# Autodesk Inventor assembly: Vacubot v1
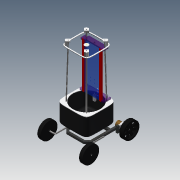
[picture p0: Inventor's stored thumbnail of the model, 180x180]
Saved by Autodesk Inventor 2014 SP1 (Build 180222100, 222)
## iProperties
Created: 2013-12-26
Part Number: Vacubot v1
Document SubType Name: Assembly
Designer: tom
Author: tom
## Documents named in this file (15)
- C:\Users\tom\Documents\GitHub\Vacubot\Inventor\Vacubot v1.iam
- C:\Users\tom\Documents\GitHub\Vacubot\Inventor\Base.ipt
- C:\Users\tom\Documents\GitHub\Vacubot\Inventor\Base Plate.ipt
- C:\Users\tom\Documents\GitHub\Vacubot\Inventor\Wheel Original.iam
- C:\Users\tom\Documents\GitHub\Vacubot\Inventor\Wheel Original_MIR.iam
- C:\Users\tom\Documents\GitHub\Vacubot\Inventor\GearMotor_Wheel.iam
- C:\Users\tom\Documents\GitHub\Vacubot\Inventor\GearMotor_Wheel_MIR.iam
- C:\Users\tom\Documents\GitHub\Vacubot\Inventor\Frame Lower.ipt
- C:\Users\tom\Documents\GitHub\Vacubot\Inventor\Part1.ipt
- C:\Users\tom\Documents\GitHub\Vacubot\Inventor\Center Rod.ipt
- C:\Users\tom\Documents\GitHub\Vacubot\Inventor\Upper Support.ipt
- C:\Users\tom\Documents\GitHub\Vacubot\Inventor\Lower Bracket.ipt
- C:\Users\tom\Documents\GitHub\Vacubot\Inventor\Gantry Motor.ipt
- C:\Users\tom\Documents\GitHub\Vacubot\Inventor\Z-table Rail.ipt
- C:\Users\tom\Documents\GitHub\Vacubot\Inventor\Z-table.ipt
## Components (18 placed, 14 different names)
1. Chassis — Mate:4, Mate:5, Mate:6
2. Base Plate:1 — Flush:1
3. Wheel Original:1 [sub-assembly]
4. Wheel Original_MIR:1 [sub-assembly]
5. GearMotor_Wheel:1 [sub-assembly] — Mate:4, Mate:5, Mate:6
6. GearMotor_Wheel_MIR:1 [sub-assembly]
7. Frame Lower:1 — Flush:1, Mate:7, Mate:8, Flush:2, Flush:5
8. Upper Chrome Frame:1 — Mate:7, Mate:8, Flush:3, Flush:4
9. Upper Bracket:1 — Flush:4, Flush:6, Mate:10, Mate:11, Mate:12, Mate:13
10. Lower Bracket:1 — Flush:5, Mate:9
11. Gantry Motor:1 — Mate:9
12. Z-table Rail:1 — Flush:6, Mate:12, Mate:13, Flush:7
13. Z-table Rail:2 — Mate:10, Mate:11
14. Z-table:1 — Flush:7
15. Center Rod:1 — Flush:2, Flush:3
16. Center Rod:2
17. Center Rod:3
18. Center Rod:4
## Component patterns: (4 elements, first: Center Rod:1)
## Relationships (20: Mate 12, Flush 7, Tangent 1)
- [Mate] (-6.35 mm): Wheel Original:1
- [Tangent]: Chassis ↔ Wheel Original:1
- [Mate] (-6.35 mm): Wheel Original:1
- Mate:4: Chassis ↔ GearMotor_Wheel:1
- Mate:5: Chassis ↔ GearMotor_Wheel:1
- Mate:6: Chassis ↔ GearMotor_Wheel:1
- Flush:1: Base Plate:1 ↔ Frame Lower:1
- Mate:7: Frame Lower:1 ↔ Upper Chrome Frame:1
- Mate:8 (304.8 mm): Frame Lower:1 ↔ Upper Chrome Frame:1
- Flush:2: Frame Lower:1 ↔ Center Rod:1
- Flush:3: Upper Chrome Frame:1 ↔ Center Rod:1
- Flush:4 (-20 mm): Upper Chrome Frame:1 ↔ Upper Bracket:1
- Flush:5 (10 mm): Frame Lower:1 ↔ Lower Bracket:1
- Mate:9: Lower Bracket:1 ↔ Gantry Motor:1
- Flush:6: Upper Bracket:1 ↔ Z-table Rail:1
- Mate:10: Upper Bracket:1 ↔ Z-table Rail:2
- Mate:11: Upper Bracket:1 ↔ Z-table Rail:2
- Mate:12: Upper Bracket:1 ↔ Z-table Rail:1
- Mate:13: Upper Bracket:1 ↔ Z-table Rail:1
- Flush:7: Z-table Rail:1 ↔ Z-table:1
